# Autodesk Inventor assembly: 付け根_1_MIR1
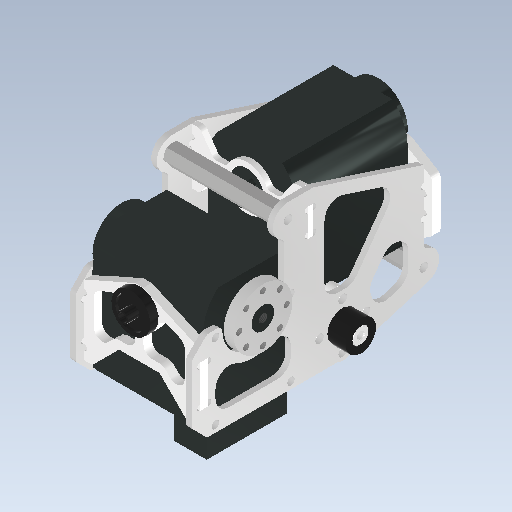
[picture p0: Inventor's stored thumbnail of the model, 512x512]
Saved by Autodesk Inventor 2020 (Build 240168000, 168)
## iProperties
Created: 2016-04-27
Part Number: 付け根_1_MIR1
Document SubType Name: Assembly
Designer: masato
Mass: 257.123 g
Surface Area: 430.699 cm^2
Volume: 127.027 cm^3
Density: 2.02416 g/cm^3
Author: hiroaki
## Documents named in this file (14)
- C:\Users\naoki\Documents\Inventor\CitBrains\git_clone\OpenPlatform167\足首再設計1\OpenPlatform_ver3_0\下半身_160823\付け根\付け根_1_MIR.iam
- C:\Users\naoki\Documents\Inventor\CitBrains\git_clone\OpenPlatform167\足首再設計1\OpenPlatform_ver3_0\既製品\free_horn.ipt
- C:\Users\naoki\Documents\Inventor\CitBrains\git_clone\OpenPlatform167\足首再設計1\OpenPlatform_ver3_0\既製品\B3M11xx.ipt
- C:\Users\naoki\Documents\Inventor\CitBrains\git_clone\OpenPlatform167\足首再設計1\OpenPlatform_ver3_0\下半身_160823\付け根\付け根_サブフレーム_1_2.ipt
- C:\Users\naoki\Documents\Inventor\CitBrains\git_clone\OpenPlatform167\足首再設計1\OpenPlatform_ver3_0\下半身\リンク\スペーサ\付け根_フリー軸_1_1.ipt
- C:\Users\naoki\Documents\Inventor\CitBrains\git_clone\OpenPlatform167\足首再設計1\OpenPlatform_ver3_0\既製品\新規購入\BRU-305_5.ipt
- C:\Users\naoki\Documents\Inventor\CitBrains\git_clone\OpenPlatform167\足首再設計1\OpenPlatform_ver3_0\下半身_160823\付け根\付け根_サブフレーム_1_4.ipt
- C:\Users\naoki\Documents\Inventor\CitBrains\git_clone\OpenPlatform167\足首再設計1\OpenPlatform_ver3_0\下半身_160823\付け根\付け根_サブフレーム_6_2.ipt
- C:\Users\naoki\Documents\Inventor\CitBrains\git_clone\OpenPlatform167\足首再設計1\OpenPlatform_ver3_0\既製品\新規購入\BRU-306_5.ipt
- C:\Users\naoki\Documents\Inventor\CitBrains\git_clone\OpenPlatform167\足首再設計1\OpenPlatform_ver3_0\下半身_160823\付け根\付け根_サブフレーム_6_4.ipt
- C:\Users\naoki\Documents\Inventor\CitBrains\git_clone\OpenPlatform167\足首再設計1\OpenPlatform_ver3_0\下半身_160823\付け根\付け根_メインフレーム_2_1.ipt
- C:\Users\naoki\Documents\Inventor\CitBrains\git_clone\OpenPlatform167\足首再設計1\OpenPlatform_ver3_0\下半身_160823\付け根\付け根_サブフレーム_1_3.ipt
- C:\Users\naoki\Documents\Inventor\CitBrains\git_clone\OpenPlatform167\足首再設計1\OpenPlatform_ver3_0\下半身_160823\付け根\付け根_メインフレーム_6_1.ipt
- C:\Users\naoki\Documents\Inventor\CitBrains\git_clone\OpenPlatform167\足首再設計1\OpenPlatform_ver3_0\既製品\SLSBF6-39_5-M3-N3.ipt
## Components (19 placed, 13 different names)
1. free_horn:1 — 挿入:1
2. B3M11xx:1 — 挿入:1, 挿入:64, 挿入:63, メイト:18, 挿入:78, 挿入:77
3. B3M11xx:2 — 挿入:8, 挿入:7, 挿入:75, 挿入:74
4. 付け根_サブフレーム_1_2:1 — 挿入:8, 挿入:7, メイト:22, フラッシュ:1, メイト:16
5. 付け根_フリー軸_1_1:1 — 挿入:66, 挿入:65
6. 付け根_フリー軸_1_1:2 — 挿入:81, 挿入:80
7. BRU-305_5:1 — 挿入:52, 挿入:76
8. 付け根_サブフレーム_1_4:1 — 挿入:82
9. 付け根_サブフレーム_6_2:1 — 挿入:52
10. BRU-306_5:1 — 挿入:55, 挿入:71
11. BRU-306_5:2 — 挿入:58
12. 付け根_サブフレーム_6_4:1 — 挿入:55
13. 付け根_サブフレーム_6_4:2 — 挿入:58, 挿入:79
14. 付け根_メインフレーム_2_1:1 — メイト:22, フラッシュ:1, メイト:16, 挿入:71, 挿入:66, 挿入:65, 挿入:64, 挿入:63, メイト:21, メイト:20, 挿入:83, 挿入:84
15. 付け根_サブフレーム_1_3:1 — 挿入:82, メイト:21, メイト:20, メイト:18
16. 付け根_メインフレーム_6_1:1 — 挿入:76, 挿入:75, 挿入:74
17. 付け根_メインフレーム_2_1:2 — 挿入:81, 挿入:80, 挿入:79, 挿入:78, 挿入:77
18. SLSBF6-39_5-M3-N3:1 — 挿入:83
19. SLSBF6-39_5-M3-N3:2 — 挿入:84
## Relationships (28: Insert 22, Mate 5, Flush 1)
- 挿入:1 [Insert]: free_horn:1 ↔ B3M11xx:1
- 挿入:8 [Insert]: B3M11xx:2 ↔ 付け根_サブフレーム_1_2:1
- 挿入:7 [Insert]: B3M11xx:2 ↔ 付け根_サブフレーム_1_2:1
- 挿入:52 [Insert]: BRU-305_5:1 ↔ 付け根_サブフレーム_6_2:1
- 挿入:55 [Insert]: BRU-306_5:1 ↔ 付け根_サブフレーム_6_4:1
- 挿入:58 [Insert]: BRU-306_5:2 ↔ 付け根_サブフレーム_6_4:2
- メイト:22 [Mate] (0.01 mm): 付け根_サブフレーム_1_2:1 ↔ 付け根_メインフレーム_2_1:1
- フラッシュ:1 [Flush]: 付け根_サブフレーム_1_2:1 ↔ 付け根_メインフレーム_2_1:1
- メイト:16 [Mate]: 付け根_サブフレーム_1_2:1 ↔ 付け根_メインフレーム_2_1:1
- 挿入:71 [Insert]: BRU-306_5:1 ↔ 付け根_メインフレーム_2_1:1
- 挿入:66 [Insert]: 付け根_フリー軸_1_1:1 ↔ 付け根_メインフレーム_2_1:1
- 挿入:65 [Insert]: 付け根_フリー軸_1_1:1 ↔ 付け根_メインフレーム_2_1:1
- 挿入:64 [Insert]: B3M11xx:1 ↔ 付け根_メインフレーム_2_1:1
- 挿入:63 [Insert]: B3M11xx:1 ↔ 付け根_メインフレーム_2_1:1
- 挿入:82 [Insert]: 付け根_サブフレーム_1_4:1 ↔ 付け根_サブフレーム_1_3:1
- メイト:21 [Mate]: 付け根_メインフレーム_2_1:1 ↔ 付け根_サブフレーム_1_3:1
- メイト:20 [Mate] (0.01 mm): 付け根_メインフレーム_2_1:1 ↔ 付け根_サブフレーム_1_3:1
- メイト:18 [Mate]: B3M11xx:1 ↔ 付け根_サブフレーム_1_3:1
- 挿入:76 [Insert]: BRU-305_5:1 ↔ 付け根_メインフレーム_6_1:1
- 挿入:75 [Insert]: B3M11xx:2 ↔ 付け根_メインフレーム_6_1:1
- 挿入:74 [Insert]: B3M11xx:2 ↔ 付け根_メインフレーム_6_1:1
- 挿入:81 [Insert]: 付け根_フリー軸_1_1:2 ↔ 付け根_メインフレーム_2_1:2
- 挿入:80 [Insert]: 付け根_フリー軸_1_1:2 ↔ 付け根_メインフレーム_2_1:2
- 挿入:79 [Insert]: 付け根_サブフレーム_6_4:2 ↔ 付け根_メインフレーム_2_1:2
- 挿入:78 [Insert]: B3M11xx:1 ↔ 付け根_メインフレーム_2_1:2
- 挿入:77 [Insert]: B3M11xx:1 ↔ 付け根_メインフレーム_2_1:2
- 挿入:83 [Insert]: 付け根_メインフレーム_2_1:1 ↔ SLSBF6-39_5-M3-N3:1
- 挿入:84 [Insert]: 付け根_メインフレーム_2_1:1 ↔ SLSBF6-39_5-M3-N3:2
